# Autodesk Inventor assembly: Wood Cutout
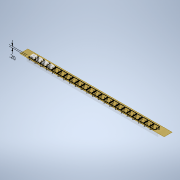
[picture p0: Inventor's stored thumbnail of the model, 180x180]
Saved by Autodesk Inventor 2022 (Build 260153000, 153)
## iProperties
Created: 2022-03-03
Part Number: Wood Cutout
Document SubType Name: Assembly
Designer: Nathan Griffith
Author: Nathan Griffith
## Documents named in this file (5)
- C:\Users\Nathan Griffith\Documents\Inventor\Eric's Keyboard\Wood Cutout.iam
- C:\Users\Nathan Griffith\Documents\Inventor\Eric's Keyboard\Stock.ipt
- C:\Users\Nathan Griffith\Documents\Inventor\Eric's Keyboard\Template Placement.ipt
- C:\Users\Nathan Griffith\Documents\Inventor\Eric's Keyboard\Keycap.ipt
- C:\Users\Nathan Griffith\Documents\Inventor\Eric's Keyboard\Bottom Holder.ipt
## Components (25 placed, 4 different names)
1. Stock:1 — Flush:1, Flush:2, Flush:3, Flush:4, Flush:5, Flush:6
2. Template Placement:1 — Flush:1, Mate:1, Mate:2, Mate:3
3. Bottom Holder:1 — Flush:2, Flush:3, Flush:4, Flush:5, Flush:6
4. Keycap:1 — Mate:1, Mate:2, Mate:3
5. Keycap:2
6. Keycap:3
7. Keycap:4
8. Keycap:5
9. Keycap:6
10. Keycap:7
11. Keycap:8
12. Keycap:9
13. Keycap:10
14. Keycap:11
15. Keycap:12
16. Keycap:13
17. Keycap:14
18. Keycap:15
19. Keycap:16
20. Keycap:17
21. Keycap:18
22. Keycap:19
23. Keycap:20
24. Keycap:21
25. Keycap:22
## Component patterns: (22 elements, first: Keycap:1)
## Relationships (9: Flush 6, Mate 3)
- Flush:1: Stock:1 ↔ Template Placement:1
- Mate:1: Template Placement:1 ↔ Keycap:1
- Mate:2: Template Placement:1 ↔ Keycap:1
- Mate:3: Template Placement:1 ↔ Keycap:1
- Flush:2: Stock:1 ↔ Bottom Holder:1
- Flush:3: Stock:1 ↔ Bottom Holder:1
- Flush:4: Stock:1 ↔ Bottom Holder:1
- Flush:5: Stock:1 ↔ Bottom Holder:1
- Flush:6: Stock:1 ↔ Bottom Holder:1
